# Autodesk Inventor assembly: batt_MIR1
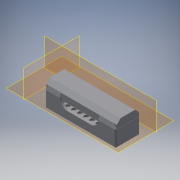
[picture p0: Inventor's stored thumbnail of the model, 180x180]
Saved by Autodesk Inventor 2016 (Build 200138000, 138)
## iProperties
Created: 2016-02-15
Part Number: batt_MIR1
Document SubType Name: Assembly
Designer: jforce
Author: jforce
## Documents named in this file (3)
- C:\Users\jforce\Dropbox\gmu\ece590 (Selective Sync Conflict)\models3\batt_MIR1.iam
- C:\Users\jforce\Dropbox\gmu\ece590 (Selective Sync Conflict)\models3\batt_cap_MIR1.ipt
- C:\Users\jforce\Dropbox\gmu\ece590 (Selective Sync Conflict)\models3\batt_carrier_MIR1.ipt
## Components (2 placed, 2 different names)
1. batt_cap_MIR1:1 — Mate:2
2. batt_carrier_MIR1:1 — Mate:2, Mate:1
## Relationships (2: Mate 2)
- Mate:2 (-6 mm): batt_cap_MIR1:1 ↔ batt_carrier_MIR1:1
- Mate:1: batt_carrier_MIR1:1
